# Autodesk Inventor assembly: manipulator
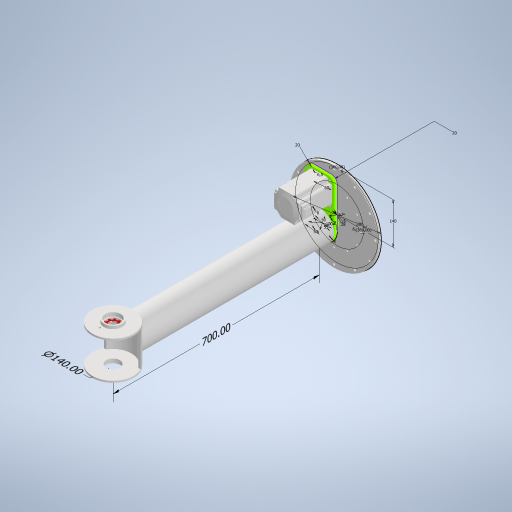
[picture p0: Inventor's stored thumbnail of the model, 512x512]
Saved by Autodesk Inventor 2023 (Build 270158000, 158)
## iProperties
Created: 2023-03-28
Part Number: manipulator
Document SubType Name: Assembly
Designer: krzys
Author: krzys
## Documents named in this file (7)
- C:\Users\Wiktor\Documents\Manipulator\Manipulator.iam
- C:\Users\Wiktor\Documents\Manipulator\podstawa.ipt
- C:\Users\Wiktor\Documents\Manipulator\manipulator\Design Accelerator\Łożysko1.iam
- C:\Users\Wiktor\Documents\Manipulator\tuleja_dystansowa.ipt
- C:\Users\Wiktor\Documents\Manipulator\podstwa_obrotowa.ipt
- C:\Users\Wiktor\Documents\Manipulator\CS-M23480_3D.ipt
- C:\Users\Wiktor\Documents\Manipulator\czlon i przekladnia.iam
## Components (7 placed, 6 different names)
1. podstawa:1
2. Łożysko:1 [sub-assembly]
3. Łożysko:2 [sub-assembly]
4. tuleja_dystansowa:1
5. podstwa_obrotowa:1 — Zestawiające:1, Zestawiające:2
6. CS-M23480_3D:1 — Zestawiające:2
7. czlon i przekladnia:1 [sub-assembly] — Zestawiające:1
## Relationships (2: Mate 2)
- Zestawiające:1 [Mate]: podstwa_obrotowa:1 ↔ czlon i przekladnia:1
- Zestawiające:2 [Mate]: podstwa_obrotowa:1 ↔ CS-M23480_3D:1
